# Autodesk Inventor assembly: Ensamblaje_Mesa
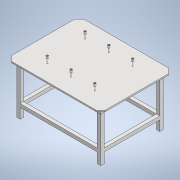
[picture p0: Inventor's stored thumbnail of the model, 180x180]
Saved by Autodesk Inventor 2021 (Build 250183000, 183)
## iProperties
Created: 2021-06-07
Part Number: Ensamblaje_Mesa
Document SubType Name: Assembly
Designer: Mecatronica
Author: Mecatronica
## Documents named in this file (3)
- G:\Unidades compartidas\Robótica\Proyecto\Ensamblaje_Mesa.iam
- G:\Unidades compartidas\Robótica\Proyecto\Mesa_Centrado.ipt
- G:\Unidades compartidas\Robótica\Proyecto\Rodillo_Sostener.ipt
## Components (7 placed, 2 different names)
1. Mesa_Centrado:1 — Coincidencia:3, Coincidencia:4, Coincidencia:5, Coincidencia:6, Coincidencia:7, Coincidencia:8, Tangente:3, Tangente:4, Tangente:6, Tangente:7, Tangente:8, Tangente:9, Tangente:10, Tangente:11, Tangente:12, Tangente:13, Tangente:14, Tangente:15
2. Rodillo_Sostener:1 — Coincidencia:7, Tangente:10, Tangente:11
3. Rodillo_Sostener:2 — Coincidencia:8, Tangente:8, Tangente:9
4. Rodillo_Sostener:3 — Coincidencia:6, Tangente:6, Tangente:7
5. Rodillo_Sostener:4 — Coincidencia:3, Tangente:3, Tangente:4
6. Rodillo_Sostener:5 — Coincidencia:5, Tangente:12, Tangente:14
7. Rodillo_Sostener:6 — Coincidencia:4, Tangente:13, Tangente:15
## Relationships (18: Tangent 12, Mate 6)
- Coincidencia:3 [Mate]: Mesa_Centrado:1 ↔ Rodillo_Sostener:4
- Coincidencia:4 [Mate]: Mesa_Centrado:1 ↔ Rodillo_Sostener:6
- Coincidencia:5 [Mate]: Mesa_Centrado:1 ↔ Rodillo_Sostener:5
- Coincidencia:6 [Mate]: Mesa_Centrado:1 ↔ Rodillo_Sostener:3
- Coincidencia:7 [Mate]: Mesa_Centrado:1 ↔ Rodillo_Sostener:1
- Coincidencia:8 [Mate]: Mesa_Centrado:1 ↔ Rodillo_Sostener:2
- Tangente:3 (344.5996 mm): Mesa_Centrado:1 ↔ Rodillo_Sostener:4
- Tangente:4 (225 mm): Mesa_Centrado:1 ↔ Rodillo_Sostener:4
- Tangente:6 (-255 mm): Mesa_Centrado:1 ↔ Rodillo_Sostener:3
- Tangente:7 (694.5561 mm): Mesa_Centrado:1 ↔ Rodillo_Sostener:3
- Tangente:8 (225 mm): Mesa_Centrado:1 ↔ Rodillo_Sostener:2
- Tangente:9 (1044.5127 mm): Mesa_Centrado:1 ↔ Rodillo_Sostener:2
- Tangente:10 (344.5996 mm): Mesa_Centrado:1 ↔ Rodillo_Sostener:1
- Tangente:11 (225 mm): Mesa_Centrado:1 ↔ Rodillo_Sostener:1
- Tangente:12 (225 mm): Mesa_Centrado:1 ↔ Rodillo_Sostener:5
- Tangente:13 (225 mm): Mesa_Centrado:1 ↔ Rodillo_Sostener:6
- Tangente:14 (694.5561 mm): Mesa_Centrado:1 ↔ Rodillo_Sostener:5
- Tangente:15 (1044.5127 mm): Mesa_Centrado:1 ↔ Rodillo_Sostener:6
